# Autodesk Inventor assembly: climber assssssembly
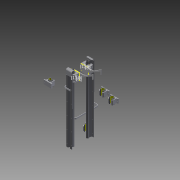
[picture p0: Inventor's stored thumbnail of the model, 180x180]
Saved by Autodesk Inventor 2013 (Build 170138000, 138)
## iProperties
Created: 2013-01-24
Part Number: climber assssssembly
Document SubType Name: Assembly
Designer: Arpan
Mass: 2447.33 g
Surface Area: 6955.59 cm^2
Volume: 1769.33 cm^3
Density: 1.3832 g/cm^3
Author: Arpan
## Documents named in this file (7)
- C:\Users\Arpan\Documents\GitHub\frc2013CAD\Climber\climber assssssembly.iam
- C:\Users\Arpan\Documents\GitHub\frc2013CAD\Climber\Shaft 26 inch.ipt
- C:\Users\Arpan\Documents\GitHub\frc2013CAD\Climber\Bearing Block long style.iam
- C:\Users\Arpan\Documents\GitHub\frc2013CAD\Climber\hook.ipt
- C:\Users\Arpan\Documents\GitHub\frc2013CAD\Climber\bearing block short style.iam
- C:\Users\Arpan\Documents\GitHub\frc2013CAD\Climber\endstop.ipt
- C:\Users\Arpan\Documents\GitHub\frc2013CAD\Climber\tie-together tier 1.ipt
## Components (14 placed, 6 different names)
1. Shaft 26 inch:1 — Angle:1, Mate:2, Angle:3, Flush:3, Mate:13, Flush:5, Mate:14, Flush:7, Mate:17, Mate:18
2. Shaft 26 inch:2 — Angle:1, Angle:2, Mate:3, Flush:3, Mate:15, Flush:6, Mate:16
3. Bearing Block long style:1 [sub-assembly] — Angle:2, Mate:3, Flush:2, Flush:4, Mate:4, Mate:8, Mate:9
4. Bearing Block long style:2 [sub-assembly] — Mate:2, Angle:3, Flush:2, Flush:4, Mate:4, Mate:5, Mate:6, Mate:7, Mate:10, Mate:11, Mate:12
5. hook:1 — Mate:5, Mate:6, Mate:7, Mate:10, Mate:11, Mate:12
6. hook:2 — Mate:8, Mate:9
7. bearing block short style:1 [sub-assembly]
8. bearing block short style:2 [sub-assembly]
9. bearing block short style:3 [sub-assembly]
10. bearing block short style:4 [sub-assembly]
11. endstop:1 — Mate:13, Flush:5, Mate:14
12. endstop:2 — Mate:15, Flush:6, Mate:16
13. tie-together tier 1:1 — Flush:7, Mate:17, Mate:18
14. tie-together tier 1:2
## Relationships (26: Mate 17, Flush 6, Angle 3)
- Angle:1 (180 deg): Shaft 26 inch:1 ↔ Shaft 26 inch:2
- Mate:2: Shaft 26 inch:1 ↔ Bearing Block long style:2
- Angle:2 (0 deg): Shaft 26 inch:2 ↔ Bearing Block long style:1
- Angle:3 (180 deg): Shaft 26 inch:1 ↔ Bearing Block long style:2
- Mate:3: Shaft 26 inch:2 ↔ Bearing Block long style:1
- Flush:2: Bearing Block long style:1 ↔ Bearing Block long style:2
- Flush:3: Shaft 26 inch:1 ↔ Shaft 26 inch:2
- Flush:4: Bearing Block long style:1 ↔ Bearing Block long style:2
- Mate:4 (88.9 mm): Bearing Block long style:1 ↔ Bearing Block long style:2
- Mate:5: Bearing Block long style:2 ↔ hook:1
- Mate:6: Bearing Block long style:2 ↔ hook:1
- Mate:7: Bearing Block long style:2 ↔ hook:1
- Mate:8: Bearing Block long style:1 ↔ hook:2
- Mate:9: Bearing Block long style:1 ↔ hook:2
- Mate:10: Bearing Block long style:2 ↔ hook:1
- Mate:11: Bearing Block long style:2 ↔ hook:1
- Mate:12: Bearing Block long style:2 ↔ hook:1
- Mate:13: Shaft 26 inch:1 ↔ endstop:1
- Flush:5: Shaft 26 inch:1 ↔ endstop:1
- Mate:14: Shaft 26 inch:1 ↔ endstop:1
- Mate:15: Shaft 26 inch:2 ↔ endstop:2
- Flush:6: Shaft 26 inch:2 ↔ endstop:2
- Mate:16: Shaft 26 inch:2 ↔ endstop:2
- Flush:7: Shaft 26 inch:1 ↔ tie-together tier 1:1
- Mate:17: Shaft 26 inch:1 ↔ tie-together tier 1:1
- Mate:18: Shaft 26 inch:1 ↔ tie-together tier 1:1
